# Autodesk Inventor assembly: ASY NDM-VOS_powder_hopper
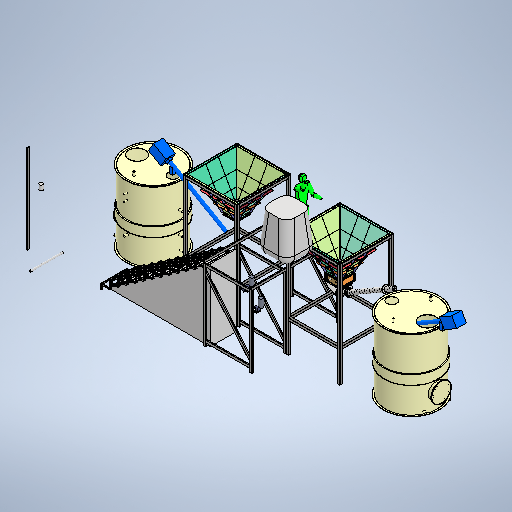
[picture p0: Inventor's stored thumbnail of the model, 512x512]
Saved by Autodesk Inventor 2025.1 (Build 291241020, 241B)
## iProperties
Created: 2024-07-24
Part Number: ASY NDM-VOS_powder_hopper
Document SubType Name: Assembly
Designer: admin
Author: admin
## Documents named in this file (27)
- C:\Users\user\YandexDisk-badmisterfox\домашниий пк\Inventor\NDM-VOS_powder_hopper\ASY NDM-VOS_powder_hopper.iam
- C:\Users\user\YandexDisk-badmisterfox\домашниий пк\Inventor\NDM-VOS_powder_hopper\Dummy 3.ipt
- C:\Users\user\YandexDisk-badmisterfox\домашниий пк\Inventor\NDM-VOS_powder_hopper\human 01\ч ASY human dummy 01.iam
- C:\Users\user\YandexDisk-badmisterfox\домашниий пк\Inventor\NDM-VOS_powder_hopper\NDM-VOS dummy3.ipt
- C:\Users\user\YandexDisk-badmisterfox\домашниий пк\Inventor\NDM-VOS_powder_hopper\NDM-VOS dummy4.ipt
- C:\Users\user\YandexDisk-badmisterfox\домашниий пк\Inventor\NDM-VOS_powder_hopper\NDM-VOS dummy5.ipt
- C:\Users\user\YandexDisk-badmisterfox\домашниий пк\Inventor\NDM-VOS_powder_hopper\NDM-VOS dummy6.ipt
- C:\Users\user\YandexDisk-badmisterfox\домашниий пк\Inventor\NDM-VOS_powder_hopper\NDM-VOS dummy FLOOR.ipt
- C:\Users\user\YandexDisk-badmisterfox\домашниий пк\Inventor\NDM-VOS_powder_hopper\NDM-VOS dummy Crane.ipt
- C:\Users\user\YandexDisk-badmisterfox\домашниий пк\Inventor\NDM-VOS_powder_hopper\NDM-VOS dummy upstairse.ipt
- C:\Users\user\YandexDisk-badmisterfox\домашниий пк\Inventor\NDM-VOS_powder_hopper\NDM-VOS 110 sheet hopper.ipt
- C:\Users\user\YandexDisk-badmisterfox\домашниий пк\Inventor\NDM-VOS_powder_hopper\Workspaces\Workspace\Cone\ASY MSC 100 cone.iam
- C:\Users\user\YandexDisk-badmisterfox\домашниий пк\Inventor\NDM-VOS_powder_hopper\ASY HPR 200  Frame.iam
- C:\Users\user\YandexDisk-badmisterfox\домашниий пк\Inventor\NDM-VOS_powder_hopper\TM06198C pump.ipt
- C:\Users\user\YandexDisk-badmisterfox\домашниий пк\Inventor\NDM-VOS_powder_hopper\ASY HPR 300 Frame human.iam
- C:\Users\user\YandexDisk-badmisterfox\домашниий пк\Inventor\NDM-VOS_powder_hopper\ASY_Ступень.iam
- C:\Users\user\YandexDisk-badmisterfox\домашниий пк\Inventor\NDM-VOS_powder_hopper\ASY стойка.iam
- C:\Users\user\YandexDisk-badmisterfox\домашниий пк\Inventor\NDM-VOS_powder_hopper\ISO 4019 - 80x40x2 - 2500.ipt
- C:\Users\user\YandexDisk-badmisterfox\домашниий пк\Inventor\NDM-VOS_powder_hopper\NVPH-401 auger.ipt
- C:\Users\user\YandexDisk-badmisterfox\домашниий пк\Inventor\NDM-VOS_powder_hopper\NVPH-402 main tube.ipt
- C:\Users\user\YandexDisk-badmisterfox\домашниий пк\Inventor\NDM-VOS_powder_hopper\NVPH-402 tube flange 1.ipt
- C:\Users\user\YandexDisk-badmisterfox\домашниий пк\Inventor\NDM-VOS_powder_hopper\NVPH-301 back side.ipt
- C:\Users\user\YandexDisk-badmisterfox\домашниий пк\Inventor\NDM-VOS_powder_hopper\NVPH-404 second tube.ipt
- C:\Users\user\YandexDisk-badmisterfox\домашниий пк\Inventor\NDM-VOS_powder_hopper\NVPH-306 front side.ipt
- C:\Users\user\YandexDisk-badmisterfox\домашниий пк\Inventor\NDM-VOS_powder_hopper\ASY NVPH-466 joint flange.iam
- C:\Users\user\YandexDisk-badmisterfox\домашниий пк\Inventor\NDM-VOS_powder_hopper\ASY NVPH-200 shredder shaft full.iam
- C:\Users\user\YandexDisk-badmisterfox\домашниий пк\Inventor\NDM-VOS_powder_hopper\NDM-VOS 111 sredder wall .ipt
## Components (52 placed, 28 different names)
1. NDM-VOS dummy3.ipt:1 — Mate:5, Mate:9
2. Dummy 3.ipt:1 — Flush:1
3. NDM-VOS dummy3.ipt:2 — Mate:6, Mate:8, Mate:9, Flush:15
4. NDM-VOS dummy4.ipt:1
5. NDM-VOS dummy5.ipt:1 — Mate:14, Flush:16
6. NDM-VOS dummy5.ipt:2 — Flush:9, Flush:15, Mate:14
7. ч ASY human dummy 01.iam:1 [sub-assembly]
8. NDM-VOS dummy6.ipt:1 — Rigid:9
9. NDM-VOS dummy FLOOR.ipt:1 — Mate:5, Mate:6, Mate:8, Mate:10, Flush:16, Mate:18
10. NDM-VOS dummy Crane.ipt:1 — Mate:10
11. NDM-VOS dummy upstairse.ipt:1 — Mate:18, Mate:23
12. NDM-VOS 110 sheet hopper.ipt:1 — Rigid:12, Rotational:10, Rotational:11
13. ASY MSC 100 cone.iam:1 [sub-assembly] — Flush:19, Mate:19, Mate:20, Rigid:9, Rigid:12, Rigid:13, Rigid:15, Rigid:16
14. ASY HPR 200  Frame.iam:1 [sub-assembly] — Flush:19, Mate:19, Mate:20, Flush:20, Flush:21, Mate:21, Rigid:3
15. TM06198C pump.ipt:1
16. ASY HPR 300 Frame human.iam:1 [sub-assembly]
17. ASY стойка.iam:1 [sub-assembly] — Flush:20, Flush:21, Mate:21, Flush:22, Flush:23, Mate:22, Rigid:5, Rigid:6
18. ASY HPR 200  Frame.iam:2 [sub-assembly] — Flush:22, Flush:23, Mate:22, Mate:26
19. ASY стойка.iam:2 [sub-assembly] — Rigid:3, Rigid:4
20. ASY стойка.iam:3 [sub-assembly] — Rigid:4, Flush:25
21. ISO 4019 - 80x40x2 - 2500.ipt:1 — Rigid:5
22. ISO 4019 - 80x40x2 - 2500.ipt:2
23. ISO 4019 - 80x40x2 - 2500.ipt:3 — Rigid:6, Flush:24, Mate:24
24. ASY MSC 100 cone.iam:2 [sub-assembly] — Mate:26
25. TM06198C pump.ipt:2
26. NVPH-401 auger.ipt:1 — Cylindrical:1
27. NVPH-402 main tube.ipt:1 — Rigid:7, Cylindrical:1, Cylindrical:2, Rigid:14, Rigid:20
28. NVPH-402 tube flange 1.ipt:1 — Rigid:7, Rotational:12
29. NVPH-301 back side.ipt:1 — Cylindrical:2, Cylindrical:3, Rigid:17
30. NVPH-404 second tube.ipt:1 — Rigid:19
31. NVPH-306 front side.ipt:1 — Cylindrical:3, Rigid:18, Flush:26
32. ASY NVPH-466 joint flange.iam:1 [sub-assembly]
33. ASY NVPH-466 joint flange.iam:2 [sub-assembly] — Rotational:12, Rigid:18
34. ASY NVPH-200 shredder shaft full.iam:1 [sub-assembly] — Rotational:10
35. ASY NVPH-200 shredder shaft full.iam:2 [sub-assembly] — Rotational:11
36. Part1:2 — Rigid:13
37. NVPH-402 tube flange 1:2 — Rigid:14
38. NDM-VOS 111 sredder wall :1 — Rigid:15, Flush:26
39. NDM-VOS 111 sredder wall :2 — Rigid:16, Rigid:17
40. NVPH-402 tube flange 1:3 — Rigid:19, Rigid:20
41. ASY_Ступень.iam:1 [sub-assembly] — Flush:24, Mate:23, Mate:24, Flush:25
42. ASY_Ступень.iam:2 [sub-assembly]
43. ASY_Ступень.iam:3 [sub-assembly]
44. ASY_Ступень.iam:4 [sub-assembly]
45. ASY_Ступень.iam:5 [sub-assembly]
46. ASY_Ступень.iam:6 [sub-assembly]
47. ASY_Ступень.iam:7 [sub-assembly]
48. ASY_Ступень.iam:8 [sub-assembly]
49. ASY_Ступень.iam:9 [sub-assembly]
50. ASY_Ступень.iam:10 [sub-assembly]
51. ASY_Ступень.iam:11 [sub-assembly]
52. ASY_Ступень.iam:12 [sub-assembly]
## Component patterns: (12 elements, first: ASY_Ступень.iam:1)
## Relationships (51: WeldJoint 16, Mate 15, Flush 13, RevoluteJoint 4, CylindricalJoint 3)
- Flush:1: Dummy 3.ipt:1
- Flush:9: NDM-VOS dummy5.ipt:2
- Mate:5: NDM-VOS dummy3.ipt:1 ↔ NDM-VOS dummy FLOOR.ipt:1
- Mate:6: NDM-VOS dummy3.ipt:2 ↔ NDM-VOS dummy FLOOR.ipt:1
- Mate:8 (1200 mm): NDM-VOS dummy3.ipt:2 ↔ NDM-VOS dummy FLOOR.ipt:1
- Mate:9 (-1830 mm): NDM-VOS dummy3.ipt:1 ↔ NDM-VOS dummy3.ipt:2
- Mate:10 (3500 mm): NDM-VOS dummy FLOOR.ipt:1 ↔ NDM-VOS dummy Crane.ipt:1
- [Mate]: NDM-VOS dummy3.ipt:2 ↔ ASY MSC 100 cone.iam:1
- Flush:15: NDM-VOS dummy3.ipt:2 ↔ NDM-VOS dummy5.ipt:2
- Mate:14: NDM-VOS dummy5.ipt:1 ↔ NDM-VOS dummy5.ipt:2
- Flush:16: NDM-VOS dummy5.ipt:1 ↔ NDM-VOS dummy FLOOR.ipt:1
- Mate:18: NDM-VOS dummy FLOOR.ipt:1 ↔ NDM-VOS dummy upstairse.ipt:1
- [Flush]: ASY HPR 200  Frame.iam:1
- Flush:19: ASY MSC 100 cone.iam:1 ↔ ASY HPR 200  Frame.iam:1
- Mate:19: ASY MSC 100 cone.iam:1 ↔ ASY HPR 200  Frame.iam:1
- Mate:20: ASY MSC 100 cone.iam:1 ↔ ASY HPR 200  Frame.iam:1
- Flush:20: ASY HPR 200  Frame.iam:1 ↔ ASY стойка.iam:1
- Flush:21: ASY HPR 200  Frame.iam:1 ↔ ASY стойка.iam:1
- Mate:21: ASY HPR 200  Frame.iam:1 ↔ ASY стойка.iam:1
- Flush:22: ASY стойка.iam:1 ↔ ASY HPR 200  Frame.iam:2
- Flush:23: ASY стойка.iam:1 ↔ ASY HPR 200  Frame.iam:2
- Mate:22: ASY стойка.iam:1 ↔ ASY HPR 200  Frame.iam:2
- Rigid:3 [WeldJoint]: ASY HPR 200  Frame.iam:1 ↔ ASY стойка.iam:2
- Rigid:4 [WeldJoint] (1000 mm): ASY стойка.iam:2 ↔ ASY стойка.iam:3
- Rigid:5 [WeldJoint]: ASY стойка.iam:1 ↔ ISO 4019 - 80x40x2 - 2500.ipt:1
- Rigid:6 [WeldJoint]: ASY стойка.iam:1 ↔ ISO 4019 - 80x40x2 - 2500.ipt:3
- Flush:24 (182 mm): ISO 4019 - 80x40x2 - 2500.ipt:3 ↔ ASY_Ступень.iam:1
- Mate:23: NDM-VOS dummy upstairse.ipt:1 ↔ ASY_Ступень.iam:1
- Mate:24: ISO 4019 - 80x40x2 - 2500.ipt:3 ↔ ASY_Ступень.iam:1
- Flush:25: ASY стойка.iam:3 ↔ ASY_Ступень.iam:1
- Mate:26: ASY HPR 200  Frame.iam:2 ↔ ASY MSC 100 cone.iam:2
- Rigid:7 [WeldJoint] (-200 mm): NVPH-402 main tube.ipt:1 ↔ NVPH-402 tube flange 1.ipt:1
- Cylindrical:1: NVPH-401 auger.ipt:1 ↔ NVPH-402 main tube.ipt:1
- Cylindrical:2: NVPH-402 main tube.ipt:1 ↔ NVPH-301 back side.ipt:1
- Rigid:9 [WeldJoint]: NDM-VOS dummy6.ipt:1 ↔ ASY MSC 100 cone.iam:1
- [WeldJoint]: NVPH-301 back side.ipt:1 ↔ ASY NVPH-466 joint flange.iam:1
- [RevoluteJoint]: NVPH-301 back side.ipt:1 ↔ ASY NVPH-466 joint flange.iam:1
- Rigid:12 [WeldJoint]: NDM-VOS 110 sheet hopper.ipt:1 ↔ ASY MSC 100 cone.iam:1
- Rotational:10 [RevoluteJoint] (-2 mm): NDM-VOS 110 sheet hopper.ipt:1 ↔ ASY NVPH-200 shredder shaft full.iam:1
- Rotational:11 [RevoluteJoint] (-2 mm): NDM-VOS 110 sheet hopper.ipt:1 ↔ ASY NVPH-200 shredder shaft full.iam:2
- Rigid:13 [WeldJoint]: ASY MSC 100 cone.iam:1 ↔ Part1:2
- Rigid:14 [WeldJoint]: NVPH-402 main tube.ipt:1 ↔ NVPH-402 tube flange 1:2
- Rotational:12 [RevoluteJoint] (-2 mm): NVPH-402 tube flange 1.ipt:1 ↔ ASY NVPH-466 joint flange.iam:2
- Rigid:15 [WeldJoint]: ASY MSC 100 cone.iam:1 ↔ NDM-VOS 111 sredder wall :1
- Rigid:16 [WeldJoint]: ASY MSC 100 cone.iam:1 ↔ NDM-VOS 111 sredder wall :2
- Cylindrical:3: NVPH-301 back side.ipt:1 ↔ NVPH-306 front side.ipt:1
- Rigid:17 [WeldJoint]: NVPH-301 back side.ipt:1 ↔ NDM-VOS 111 sredder wall :2
- Rigid:18 [WeldJoint]: NVPH-306 front side.ipt:1 ↔ ASY NVPH-466 joint flange.iam:2
- Flush:26: NVPH-306 front side.ipt:1 ↔ NDM-VOS 111 sredder wall :1
- Rigid:19 [WeldJoint]: NVPH-404 second tube.ipt:1 ↔ NVPH-402 tube flange 1:3
- Rigid:20 [WeldJoint] (-2 mm): NVPH-402 main tube.ipt:1 ↔ NVPH-402 tube flange 1:3
